# Autodesk Inventor assembly: TiltMountExShort
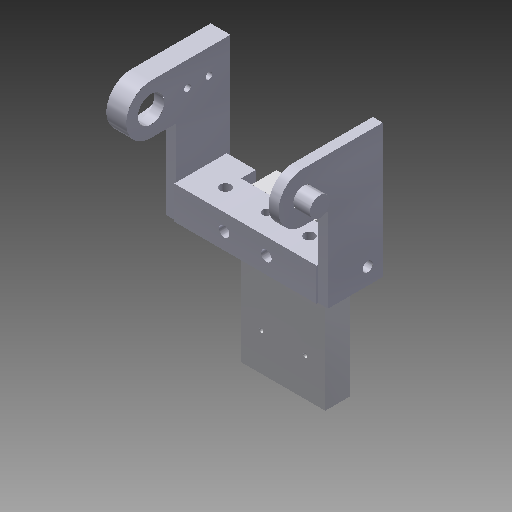
[picture p0: Inventor's stored thumbnail of the model, 512x512]
Saved by Autodesk Inventor 2017 (Build 210142000, 142)
## iProperties
Created: 2017-03-21
Part Number: TiltMountExShort
Document SubType Name: Assembly
Designer: Naga
Author: Naga
## Documents named in this file (5)
- E:\GDrive\IEEE CS\SoutheastCon2017\Cad\tilt\TiltMountExShort.iam
- E:\GDrive\IEEE CS\SoutheastCon2017\Cad\tilt\exBase.ipt
- E:\GDrive\IEEE CS\SoutheastCon2017\Cad\tilt\exShort.ipt
- E:\GDrive\IEEE CS\SoutheastCon2017\Cad\tilt\exShortShaft.ipt
- E:\GDrive\IEEE CS\SoutheastCon2017\Cad\tilt\magMount.ipt
## Components (4 placed, 4 different names)
1. exBase:1 — Mate:1, Mate:2, Flush:1, Flush:2, Mate:3, Mate:4, Mate:5, Flush:3, Mate:6
2. exShort:1 — Mate:1, Mate:2, Flush:1
3. exShortShaft:1 — Flush:2, Mate:3, Mate:4
4. magMount:1 — Mate:5, Flush:3, Mate:6
## Relationships (9: Mate 6, Flush 3)
- Mate:1: exBase:1 ↔ exShort:1
- Mate:2: exBase:1 ↔ exShort:1
- Flush:1: exBase:1 ↔ exShort:1
- Flush:2: exBase:1 ↔ exShortShaft:1
- Mate:3: exBase:1 ↔ exShortShaft:1
- Mate:4: exBase:1 ↔ exShortShaft:1
- Mate:5: exBase:1 ↔ magMount:1
- Flush:3: exBase:1 ↔ magMount:1
- Mate:6: exBase:1 ↔ magMount:1
